# Autodesk Inventor assembly: Assembly1
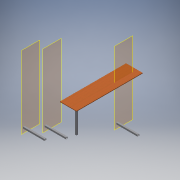
[picture p0: Inventor's stored thumbnail of the model, 180x180]
Saved by Autodesk Inventor 2016 (Build 200138000, 138)
## iProperties
Created: 2018-06-24
Part Number: Assembly1
Document SubType Name: Assembly
Designer: damia
Author: damia
## Documents named in this file (3)
- C:\Users\damia\Documents\Inventor\escritorio_Damian\Assembly1.iam
- C:\Users\damia\Documents\Inventor\escritorio_Damian\tablero_mesada.ipt
- C:\Users\damia\Documents\Inventor\escritorio_Damian\Pata.ipt
## Components (5 placed, 2 different names)
1. tablero_mesada:1 — Flush:1, Mate:1, Flush:2, Flush:3
2. Pata:1 — Flush:2, Flush:3
3. Pata:2
4. Pata:3
5. Pata:4
## Relationships (4: Flush 3, Mate 1)
- Flush:1: tablero_mesada:1
- Mate:1: tablero_mesada:1
- Flush:2: tablero_mesada:1 ↔ Pata:1
- Flush:3: tablero_mesada:1 ↔ Pata:1
